# Autodesk Inventor assembly: lan26-160_silder_pan26-3_Rails_Assembly_Rev2
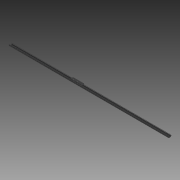
[picture p0: Inventor's stored thumbnail of the model, 180x180]
Saved by Autodesk Inventor 2015 (Build 190159000, 159)
## iProperties
Created: 2016-12-23
Part Number: lan26-160_silder_pan26-3_Rails_Assembly_Rev2
Document SubType Name: Assembly
Designer: Guy
Author: Guy
## Documents named in this file (3)
- C:\Users\Ernest\Documents\Capstone-Project\doc\CAD\Rails CAD\lan26-160_silder_pan26-3_Rails_Assembly_Rev2.iam
- C:\Users\Ernest\Documents\Capstone-Project\doc\CAD\Rails CAD\lan26-160 Inventor\rail_lan26-160.ipt
- C:\Users\Ernest\Documents\Capstone-Project\doc\CAD\Rails CAD\slider_pan26-3 Inventor\slider_pan26-3.ipt
## Components (2 placed, 2 different names)
1. rail_lan26-160:1 — Mate:1, Tangent:1, Tangent:2
2. slider_pan26-3:1 — Mate:1, Tangent:1, Tangent:2
## Relationships (3: Tangent 2, Mate 1)
- Mate:1: rail_lan26-160:1 ↔ slider_pan26-3:1
- Tangent:1: rail_lan26-160:1 ↔ slider_pan26-3:1
- Tangent:2: rail_lan26-160:1 ↔ slider_pan26-3:1
